# Autodesk Inventor assembly: Shoter_4
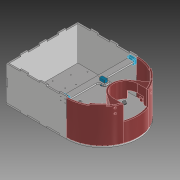
[picture p0: Inventor's stored thumbnail of the model, 180x180]
Saved by Autodesk Inventor 2022 (Build 260153000, 153)
## iProperties
Created: 2025-01-23
Part Number: Shoter_4
Document SubType Name: Assembly
Designer: Ivan
Author: Ivan
## Documents named in this file (13)
- E:\4. Прочее\1517\Предпрофессиональная олимпиада\Shoter_V4\Shoter_4_Res\Корпус.iam
- E:\4. Прочее\1517\Предпрофессиональная олимпиада\Shoter_V4\Корпус\Основание нижнее.ipt
- E:\4. Прочее\1517\Предпрофессиональная олимпиада\Shoter_V4\Корпус\Кронштейн сервопривода.ipt
- E:\4. Прочее\1517\Предпрофессиональная олимпиада\Shoter_V4\Корпус\Стенка боковая.ipt
- E:\4. Прочее\1517\Предпрофессиональная олимпиада\Shoter_V4\Корпус\Стенка задняя.ipt
- E:\4. Прочее\1517\Предпрофессиональная олимпиада\Shoter_V4\Корпус\Кожух левый.ipt
- E:\4. Прочее\1517\Предпрофессиональная олимпиада\Shoter_V4\Корпус\Кожух малый.ipt
- E:\4. Прочее\1517\Предпрофессиональная олимпиада\Shoter_V4\Корпус\Кожух правый.ipt
- E:\4. Прочее\1517\Предпрофессиональная олимпиада\Shoter_V4\Корпус\Кожухзадний.ipt
- E:\4. Прочее\1517\Предпрофессиональная олимпиада\Shoter_V4\Фиксатор_сервопривода.ipt
- E:\4. Прочее\1517\Предпрофессиональная олимпиада\Shoter_V4\SG90.ipt
- E:\4. Прочее\1517\Предпрофессиональная олимпиада\Shoter_V4\Упор_В2.ipt
- C:\Школа\1517_Предпроф_2024-2025\Наливатор_акт\Shoter_1_ZIP\1.ipt
## Components (17 placed, 12 different names)
1. Основание нижнее:1 — Совмещение:1, Заподлицо:1, Заподлицо:2, Совмещение:2, Заподлицо:3, Заподлицо:5, Совмещение:3, Совмещение:4, Совмещение:5, Совмещение:6, Совмещение:7, Совмещение:11, Совмещение:27, Совмещение:28, Совмещение:29, Совмещение:30, Совмещение:31, Совмещение:32
2. Кронштейн сервопривода:1 — Совмещение:12, Совмещение:19, Совмещение:20, Совмещение:24, Совмещение:25, Совмещение:26
3. Стенка боковая:1 — Совмещение:1, Заподлицо:1, Заподлицо:2, Заподлицо:4, Совмещение:9, Совмещение:12, Совмещение:13, Совмещение:14, Совмещение:15
4. Стенка задняя:1 — Совмещение:2, Заподлицо:3, Заподлицо:4, Заподлицо:6, Заподлицо:7
5. Кожух левый:1 — Совмещение:3, Совмещение:6, Совмещение:8, Совмещение:10, Совмещение:21, Совмещение:22, Совмещение:33
6. Кожух малый:1 — Совмещение:5, Совмещение:10, Совмещение:11
7. Кожух правый:1 — Совмещение:4, Совмещение:7, Совмещение:9, Совмещение:23
8. Кожухзадний:1 — Совмещение:21, Совмещение:22, Совмещение:23
9. Стенка боковая:2 — Заподлицо:5, Заподлицо:6, Заподлицо:7, Совмещение:8, Совмещение:16, Совмещение:17, Совмещение:18
10. Фиксатор_сервопривода:1 — Совмещение:13, Совмещение:14, Совмещение:15, Совмещение:20
11. Фиксатор_сервопривода:2 — Совмещение:16, Совмещение:17, Совмещение:18, Совмещение:19
12. SG90:1 — Совмещение:24, Совмещение:25, Совмещение:26
13. Упор_В2:1 — Совмещение:27, Совмещение:28, Заподлицо:8, Заподлицо:9
14. Упор_В2:2 — Совмещение:29, Заподлицо:9, Заподлицо:10
15. Упор_В2:3 — Совмещение:30, Заподлицо:10
16. Упор_В2:4 — Совмещение:31, Заподлицо:8
17. 1:1 — Совмещение:32, Совмещение:33, Заподлицо:11
## Relationships (44: Mate 33, Flush 11)
- Совмещение:1 [Mate]: Основание нижнее:1 ↔ Стенка боковая:1
- Заподлицо:1 [Flush]: Основание нижнее:1 ↔ Стенка боковая:1
- Заподлицо:2 [Flush]: Основание нижнее:1 ↔ Стенка боковая:1
- Совмещение:2 [Mate]: Основание нижнее:1 ↔ Стенка задняя:1
- Заподлицо:3 [Flush]: Основание нижнее:1 ↔ Стенка задняя:1
- Заподлицо:4 [Flush]: Стенка боковая:1 ↔ Стенка задняя:1
- Заподлицо:5 [Flush]: Основание нижнее:1 ↔ Стенка боковая:2
- Заподлицо:6 [Flush]: Стенка задняя:1 ↔ Стенка боковая:2
- Заподлицо:7 [Flush]: Стенка задняя:1 ↔ Стенка боковая:2
- Совмещение:3 [Mate]: Основание нижнее:1 ↔ Кожух левый:1
- Совмещение:4 [Mate]: Основание нижнее:1 ↔ Кожух правый:1
- Совмещение:5 [Mate]: Основание нижнее:1 ↔ Кожух малый:1
- Совмещение:6 [Mate]: Основание нижнее:1 ↔ Кожух левый:1
- Совмещение:7 [Mate]: Основание нижнее:1 ↔ Кожух правый:1
- Совмещение:8 [Mate]: Кожух левый:1 ↔ Стенка боковая:2
- Совмещение:9 [Mate]: Стенка боковая:1 ↔ Кожух правый:1
- Совмещение:10 [Mate]: Кожух левый:1 ↔ Кожух малый:1
- Совмещение:11 [Mate]: Основание нижнее:1 ↔ Кожух малый:1
- Совмещение:12 [Mate]: Кронштейн сервопривода:1 ↔ Стенка боковая:1
- Совмещение:13 [Mate]: Стенка боковая:1 ↔ Фиксатор_сервопривода:1
- Совмещение:14 [Mate]: Стенка боковая:1 ↔ Фиксатор_сервопривода:1
- Совмещение:15 [Mate]: Стенка боковая:1 ↔ Фиксатор_сервопривода:1
- Совмещение:16 [Mate]: Стенка боковая:2 ↔ Фиксатор_сервопривода:2
- Совмещение:17 [Mate]: Стенка боковая:2 ↔ Фиксатор_сервопривода:2
- Совмещение:18 [Mate]: Стенка боковая:2 ↔ Фиксатор_сервопривода:2
- Совмещение:19 [Mate]: Кронштейн сервопривода:1 ↔ Фиксатор_сервопривода:2
- Совмещение:20 [Mate]: Кронштейн сервопривода:1 ↔ Фиксатор_сервопривода:1
- Совмещение:21 [Mate]: Кожух левый:1 ↔ Кожухзадний:1
- Совмещение:22 [Mate]: Кожух левый:1 ↔ Кожухзадний:1
- Совмещение:23 [Mate]: Кожух правый:1 ↔ Кожухзадний:1
- Совмещение:24 [Mate]: Кронштейн сервопривода:1 ↔ SG90:1
- Совмещение:25 [Mate]: Кронштейн сервопривода:1 ↔ SG90:1
- Совмещение:26 [Mate]: Кронштейн сервопривода:1 ↔ SG90:1
- Совмещение:27 [Mate]: Основание нижнее:1 ↔ Упор_В2:1
- Совмещение:28 [Mate]: Основание нижнее:1 ↔ Упор_В2:1
- Совмещение:29 [Mate]: Основание нижнее:1 ↔ Упор_В2:2
- Совмещение:30 [Mate]: Основание нижнее:1 ↔ Упор_В2:3
- Совмещение:31 [Mate]: Основание нижнее:1 ↔ Упор_В2:4
- Заподлицо:8 [Flush]: Упор_В2:1 ↔ Упор_В2:4
- Заподлицо:9 [Flush]: Упор_В2:1 ↔ Упор_В2:2
- Заподлицо:10 [Flush]: Упор_В2:2 ↔ Упор_В2:3
- Совмещение:32 [Mate]: Основание нижнее:1 ↔ 1:1
- Совмещение:33 [Mate]: Кожух левый:1 ↔ 1:1
- Заподлицо:11 [Flush]: 1:1
